# Autodesk Inventor assembly: ASY фильтр пакет
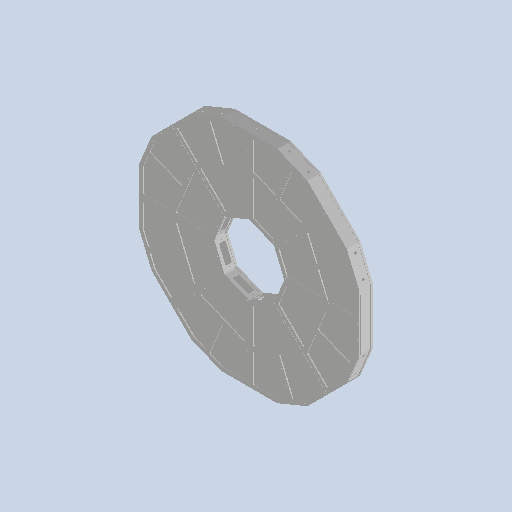
[picture p0: Inventor's stored thumbnail of the model, 512x512]
Saved by Autodesk Inventor 2025 (Build 290162010, 162A)
## iProperties
Created: 2024-05-16
Part Number: ASY фильтр пакет
Document SubType Name: Assembly
Designer: admin
Author: admin
## Documents named in this file (2)
- C:\Users\pokla\Documents\Inventor\ДФО\ДМФ\DMF-Disk-Micro-Filter\ASY фильтр пакет.iam
- C:\Users\pokla\Documents\Inventor\ДФО\ДМФ\DMF-Disk-Micro-Filter\ASY ДМФ 01 50 Кассета.iam
## Components (8 placed, 1 different names)
1. ASY ДМФ 01 50 Кассета:1 [sub-assembly] — Mate:1, Flush:1
2. ASY ДМФ 01 50 Кассета:2 [sub-assembly]
3. ASY ДМФ 01 50 Кассета:3 [sub-assembly] — Flush:2
4. ASY ДМФ 01 50 Кассета:4 [sub-assembly]
5. ASY ДМФ 01 50 Кассета:5 [sub-assembly]
6. ASY ДМФ 01 50 Кассета:6 [sub-assembly]
7. ASY ДМФ 01 50 Кассета:7 [sub-assembly]
8. ASY ДМФ 01 50 Кассета:8 [sub-assembly]
## Relationships (10: WeldJoint 7, Flush 2, Mate 1)
- [WeldJoint]: ASY ДМФ 01 50 Кассета:1 ↔ ASY ДМФ 01 50 Кассета:2
- [WeldJoint]: ASY ДМФ 01 50 Кассета:2 ↔ ASY ДМФ 01 50 Кассета:3
- [WeldJoint]: ASY ДМФ 01 50 Кассета:3 ↔ ASY ДМФ 01 50 Кассета:4
- [WeldJoint]: ASY ДМФ 01 50 Кассета:4 ↔ ASY ДМФ 01 50 Кассета:5
- [WeldJoint]: ASY ДМФ 01 50 Кассета:5 ↔ ASY ДМФ 01 50 Кассета:6
- [WeldJoint]: ASY ДМФ 01 50 Кассета:6 ↔ ASY ДМФ 01 50 Кассета:7
- [WeldJoint]: ASY ДМФ 01 50 Кассета:7 ↔ ASY ДМФ 01 50 Кассета:8
- Mate:1: ASY ДМФ 01 50 Кассета:1
- Flush:1: ASY ДМФ 01 50 Кассета:1
- Flush:2: ASY ДМФ 01 50 Кассета:3
